# Autodesk Inventor assembly: Zusammenbau Feder Topf
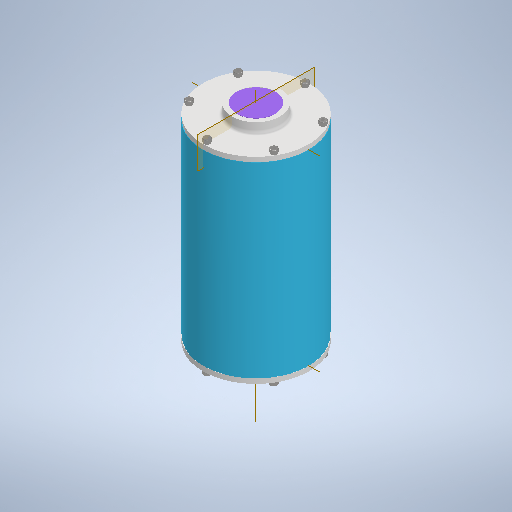
[picture p0: Inventor's stored thumbnail of the model, 512x512]
Saved by Autodesk Inventor 2025.2 (Build 292293000, 293)
## iProperties
Created: 2022-11-23
Part Number: Zusammenbau Feder Topf
Document SubType Name: Assembly
Designer: schil
Author: schil
## Documents named in this file (9)
- \\Mac\Dokumente\CAD_Test\Eingangs- und Abschlusstest\Zusammenbau Feder Topf.iam
- \\Mac\Dokumente\CAD_Test\Eingangs- und Abschlusstest\Deckel Stempel.ipt
- \\Mac\Dokumente\CAD_Test\Eingangs- und Abschlusstest\Stempel.ipt
- \\Mac\Dokumente\CAD_Test\Eingangs- und Abschlusstest\Gehaeuse.ipt
- \\Mac\Dokumente\CAD_Test\Eingangs- und Abschlusstest\Deckel Stempel 2.ipt
- \\Mac\Dokumente\CAD_Test\Eingangs- und Abschlusstest\Compress Spring11.ipt
- \\Mac\Dokumente\CAD_Test\Eingangs- und Abschlusstest\Topf.ipt
- \\Mac\Dokumente\CAD_Test\Eingangs- und Abschlusstest\Compress Spring12.ipt
- C:\Users\tino\Documents_VM\Inventor\Content Center Files\R2025\de-DE\ISO 4762(2)\ISO 4762 - M4 x 10ISO.ipt
## Components (21 placed, 7 different names)
1. Deckel Stempel:1 — Passend:1, Passend:4, Passend:5, Passend:6, Passend:7, Einfügen:8, Einfügen:9, Einfügen:10, Einfügen:11, Einfügen:12, Einfügen:13
2. Stempel:1 — Passend:1, Passend:4, Passend:17, Passend:18
3. Gehaeuse:1 — Passend:5, Passend:6, Passend:7, Passend:13, Passend:14
4. ISO 4762 M4 x 10:1
5. ISO 4762 M4 x 10:9
6. Deckel Stempel 2:1 — Passend:13, Passend:14
7. Compress Spring1:1 — Passend:17, Passend:18, Passend:19, Passend:20, Passend:22
8. Topf:1 — Passend:19, Passend:20, Passend:21
9. Compress Spring1:1 — Passend:21, Passend:22
10. ISO 4762 M4 x 10:23 — Einfügen:8
11. ISO 4762 M4 x 10:24 — Einfügen:9
12. ISO 4762 M4 x 10:25 — Einfügen:10
13. ISO 4762 M4 x 10:26 — Einfügen:11
14. ISO 4762 M4 x 10:27 — Einfügen:12
15. ISO 4762 M4 x 10:28 — Einfügen:13
16. ISO 4762 M4 x 10:10
17. ISO 4762 M4 x 10:11
18. ISO 4762 M4 x 10:12
19. ISO 4762 M4 x 10:13
20. ISO 4762 M4 x 10:14
21. ISO 4762 M4 x 10:15
## Component patterns: (6 elements, first: ISO 4762 M4 x 10:10)
## Relationships (25: Mate 19, Insert 6)
- Passend:1 [Mate]: Deckel Stempel:1 ↔ Stempel:1
- Passend:4 [Mate]: Deckel Stempel:1 ↔ Stempel:1
- Passend:5 [Mate]: Deckel Stempel:1 ↔ Gehaeuse:1
- Passend:6 [Mate]: Deckel Stempel:1 ↔ Gehaeuse:1
- Passend:7 [Mate]: Deckel Stempel:1 ↔ Gehaeuse:1
- [Mate]: Deckel Stempel:1 ↔ ISO 4762 M4 x 10:1
- [Mate]: Deckel Stempel:1 ↔ ISO 4762 M4 x 10:1
- [Mate]: Deckel Stempel:1 ↔ ISO 4762 M4 x 10:9
- [Mate]: Deckel Stempel:1 ↔ ISO 4762 M4 x 10:9
- Passend:13 [Mate]: Gehaeuse:1 ↔ Deckel Stempel 2:1
- Passend:14 [Mate]: Gehaeuse:1 ↔ Deckel Stempel 2:1
- [Mate]: Deckel Stempel 2:1 ↔ ISO 4762 M4 x 10:10
- [Mate]: Deckel Stempel 2:1 ↔ ISO 4762 M4 x 10:10
- Passend:17 [Mate]: Stempel:1 ↔ Compress Spring1:1
- Passend:18 [Mate]: Stempel:1 ↔ Compress Spring1:1
- Passend:19 [Mate]: Compress Spring1:1 ↔ Topf:1
- Passend:20 [Mate]: Compress Spring1:1 ↔ Topf:1
- Passend:21 [Mate]: Topf:1 ↔ Compress Spring1:1
- Passend:22 [Mate]: Compress Spring1:1
- Einfügen:8 [Insert]: Deckel Stempel:1 ↔ ISO 4762 M4 x 10:23
- Einfügen:9 [Insert]: Deckel Stempel:1 ↔ ISO 4762 M4 x 10:24
- Einfügen:10 [Insert]: Deckel Stempel:1 ↔ ISO 4762 M4 x 10:25
- Einfügen:11 [Insert]: Deckel Stempel:1 ↔ ISO 4762 M4 x 10:26
- Einfügen:12 [Insert]: Deckel Stempel:1 ↔ ISO 4762 M4 x 10:27
- Einfügen:13 [Insert]: Deckel Stempel:1 ↔ ISO 4762 M4 x 10:28
